# Autodesk Inventor assembly: AssemblyRespiratoriam
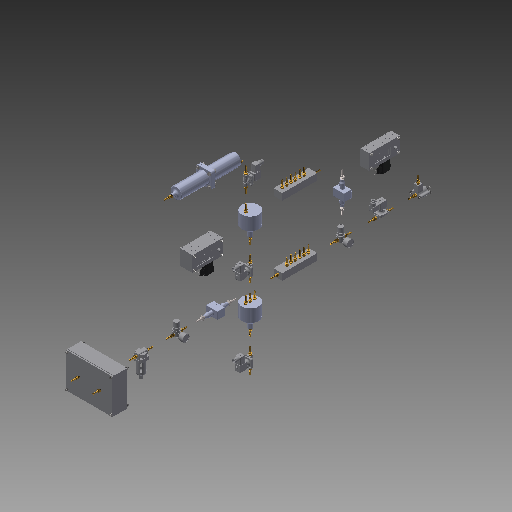
[picture p0: Inventor's stored thumbnail of the model, 512x512]
Saved by Autodesk Inventor 2018 (Build 220112000, 112)
## iProperties
Created: 2020-03-29
Part Number: AssemblyRespiratoriam
Document SubType Name: Assembly
Designer: emile
Author: emile
## Documents named in this file (12)
- C:\Users\emile\OneDrive\Documents\GitHub\VentilatorCovid19\Respirator\MultiLine\AssemblyRespiratoriam.iam
- C:\Users\emile\OneDrive\Documents\GitHub\VentilatorCovid19\Respirator\MultiLine\SolenoidValve.iam
- C:\Users\emile\OneDrive\Documents\GitHub\VentilatorCovid19\Respirator\MultiLine\Air filter.iam
- C:\Users\emile\OneDrive\Documents\GitHub\VentilatorCovid19\Respirator\MultiLine\Pressure regulator.iam
- C:\Users\emile\OneDrive\Documents\GitHub\VentilatorCovid19\Respirator\MultiLine\WaterOilSeparator.iam
- C:\Users\emile\OneDrive\Documents\GitHub\VentilatorCovid19\Respirator\MultiLine\SplitterBlock.iam
- C:\Users\emile\OneDrive\Documents\GitHub\VentilatorCovid19\Respirator\Peep\AirPressure\PeepVavle.iam
- C:\Users\emile\OneDrive\Documents\GitHub\VentilatorCovid19\Respirator\MultiLine\ArduinoCase\CaseAssembly.iam
- C:\Users\emile\OneDrive\Documents\GitHub\VentilatorCovid19\Respirator\MultiLine\MedicalAirFilter\Medical Air Filter Assy (1).iam
- C:\Users\emile\OneDrive\Documents\GitHub\VentilatorCovid19\Respirator\MultiLine\Humidificator\Humidifier Assembly.iam
- C:\Users\emile\OneDrive\Documents\GitHub\VentilatorCovid19\Respirator\MultiLine\ArduinoCase\CaseBoilerAssembly.iam
- C:\Users\emile\OneDrive\Documents\GitHub\VentilatorCovid19\Respirator\MultiLine\boiler\Boiler-SubAssy.iam
## Components (14 placed, 11 different names)
1. SolenoidValve:1 [sub-assembly] — Mate:3, Angle:3, Mate:8, Mate:9, Mate:13, Mate:14
2. Air filter:1 [sub-assembly] — Mate:4, Mate:6, Angle:5, Mate:24
3. Pressure regulator:1 [sub-assembly] — Mate:2, Mate:3, Flush:1, Flush:2, Mate:7, Mate:8
4. WaterOilSeparator:1 [sub-assembly] — Mate:1, Mate:4, Angle:2, Mate:6, Mate:12
5. SplitterBlock:1 [sub-assembly] — Mate:1, Mate:2, Angle:1, Mate:7, Mate:11, Flush:3, Angle:7, Mate:15, Mate:19, Flush:8, Flush:9
6. PeepVavle:1 [sub-assembly] — Mate:9, Angle:4, Mate:21
7. Pressure regulator:2 [sub-assembly] — Mate:11, Angle:6, Mate:12, Mate:16
8. CaseAssembly:1 [sub-assembly] — Flush:3, Angle:7, Mate:13, Mate:14, Flush:4, Flush:5
9. Medical Air Filter Assy (1):1 [sub-assembly] — Mate:15, Angle:8, Mate:16, Mate:17, Mate:18, Mate:20, Flush:6
10. Humidifier Assembly:1 [sub-assembly] — Mate:17, Mate:18, Mate:19, Mate:20, Mate:22, Mate:23
11. CaseBoilerAssembly:1 [sub-assembly] — Flush:4, Flush:5, Flush:6
12. Boiler-SubAssy:1 [sub-assembly] — Mate:21, Mate:22, Mate:23
13. SplitterBlock:2 [sub-assembly] — Flush:8, Flush:9, Mate:25
14. Medical Air Filter Assy (1):2 [sub-assembly] — Mate:24, Mate:25
## Relationships (39: Mate 23, Flush 8, Angle 8)
- Mate:1: WaterOilSeparator:1 ↔ SplitterBlock:1
- Mate:2: Pressure regulator:1 ↔ SplitterBlock:1
- Mate:3: SolenoidValve:1 ↔ Pressure regulator:1
- Mate:4: Air filter:1 ↔ WaterOilSeparator:1
- Flush:1: Pressure regulator:1
- Flush:2: Pressure regulator:1
- Angle:1 (0 deg): SplitterBlock:1
- Angle:2 (0 deg): WaterOilSeparator:1
- Angle:3 (0 deg): SolenoidValve:1
- Mate:6 (101.6 mm): Air filter:1 ↔ WaterOilSeparator:1
- Mate:7 (101.6 mm): Pressure regulator:1 ↔ SplitterBlock:1
- Mate:8 (101.6 mm): SolenoidValve:1 ↔ Pressure regulator:1
- Mate:9: SolenoidValve:1 ↔ PeepVavle:1
- Angle:4 (180 deg): PeepVavle:1
- Angle:5 (0 deg): Air filter:1
- Mate:11: SplitterBlock:1 ↔ Pressure regulator:2
- Angle:6 (0 deg): Pressure regulator:2
- Mate:12 (76.2 mm): WaterOilSeparator:1 ↔ Pressure regulator:2
- Flush:3: SplitterBlock:1 ↔ CaseAssembly:1
- Angle:7 (180 deg): SplitterBlock:1 ↔ CaseAssembly:1
- Mate:13 (203.2 mm): SolenoidValve:1 ↔ CaseAssembly:1
- Mate:14: SolenoidValve:1 ↔ CaseAssembly:1
- Mate:15: SplitterBlock:1 ↔ Medical Air Filter Assy (1):1
- Angle:8 (0 deg): Medical Air Filter Assy (1):1
- Mate:16 (50.8 mm): Pressure regulator:2 ↔ Medical Air Filter Assy (1):1
- Mate:17: Medical Air Filter Assy (1):1 ↔ Humidifier Assembly:1
- Mate:18: Medical Air Filter Assy (1):1 ↔ Humidifier Assembly:1
- Mate:19 (101.6 mm): SplitterBlock:1 ↔ Humidifier Assembly:1
- Mate:20 (101.6 mm): Medical Air Filter Assy (1):1 ↔ Humidifier Assembly:1
- Flush:4: CaseAssembly:1 ↔ CaseBoilerAssembly:1
- Flush:5: CaseAssembly:1 ↔ CaseBoilerAssembly:1
- Flush:6: Medical Air Filter Assy (1):1 ↔ CaseBoilerAssembly:1
- Mate:21: PeepVavle:1 ↔ Boiler-SubAssy:1
- Mate:22 (50.8 mm): Humidifier Assembly:1 ↔ Boiler-SubAssy:1
- Mate:23 (76.2 mm): Humidifier Assembly:1 ↔ Boiler-SubAssy:1
- Flush:8: SplitterBlock:1 ↔ SplitterBlock:2
- Flush:9: SplitterBlock:1 ↔ SplitterBlock:2
- Mate:24: Air filter:1 ↔ Medical Air Filter Assy (1):2
- Mate:25 (25.4 mm): SplitterBlock:2 ↔ Medical Air Filter Assy (1):2
